# Autodesk Inventor assembly: TopAssembly
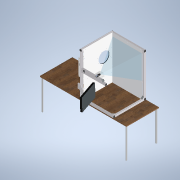
[picture p0: Inventor's stored thumbnail of the model, 180x180]
Saved by Autodesk Inventor 2020 (Build 240168000, 168)
## iProperties
Created: 2019-11-06
Part Number: TopAssembly
Document SubType Name: Assembly
Designer: nicoc
Author: nicoc
## Documents named in this file (9)
- D:\Repos\P5-AIonFPGA\cad\TopAssembly.iam
- D:\Repos\P5-AIonFPGA\cad\BasicFramework\BasicFramework.iam
- D:\Repos\P5-AIonFPGA\cad\RearPanel\RearPanel.iam
- D:\Repos\P5-AIonFPGA\cad\SidePanel\SidePanel.iam
- D:\Repos\P5-AIonFPGA\cad\Cameramounting\Cameramounting.iam
- D:\Repos\P5-AIonFPGA\cad\Table\Table.iam
- D:\Repos\P5-AIonFPGA\cad\Display\Display.iam
- D:\Repos\P5-AIonFPGA\cad\Case\Case.iam
- D:\Repos\P5-AIonFPGA\cad\Lighting\LHF300\LHF300-R2.iam
## Components (8 placed, 8 different names)
1. BasicFramework:1 [sub-assembly] — Mate:1, Flush:1, Mate:2, Mate:5, Flush:3, Mate:6, Mate:7, Flush:4, Flush:5, Mate:8, Mate:10, Flush:7, Mate:17, Flush:9, Mate:18, Flush:11
2. RearPanel:1 [sub-assembly] — Mate:1, Flush:1, Mate:2, Mate:11, Mate:14
3. SidePanel:1 [sub-assembly] — Mate:10, Flush:7, Mate:11
4. Cameramounting:1 [sub-assembly] — Mate:5, Flush:3, Mate:6, Flush:10
5. Table:1 [sub-assembly] — Mate:7, Flush:4, Flush:5
6. Display:1 [sub-assembly] — Mate:8, Mate:17, Flush:9
7. Case:1 [sub-assembly] — Mate:14
8. LHF300-R2:1 [sub-assembly] — Flush:10, Mate:18, Flush:11
## Relationships (19: Mate 11, Flush 8)
- Mate:1: BasicFramework:1 ↔ RearPanel:1
- Flush:1: BasicFramework:1 ↔ RearPanel:1
- Mate:2 (0.5 mm): BasicFramework:1 ↔ RearPanel:1
- Mate:5: BasicFramework:1 ↔ Cameramounting:1
- Flush:3: BasicFramework:1 ↔ Cameramounting:1
- Mate:6 (-664.5 mm): BasicFramework:1 ↔ Cameramounting:1
- Mate:7: BasicFramework:1 ↔ Table:1
- Flush:4: BasicFramework:1 ↔ Table:1
- Flush:5 (-300 mm): BasicFramework:1 ↔ Table:1
- Mate:8: BasicFramework:1 ↔ Display:1
- Mate:10: BasicFramework:1 ↔ SidePanel:1
- Flush:7: BasicFramework:1 ↔ SidePanel:1
- Mate:11: RearPanel:1 ↔ SidePanel:1
- Mate:14 (5 mm): RearPanel:1 ↔ Case:1
- Mate:17: BasicFramework:1 ↔ Display:1
- Flush:9: BasicFramework:1 ↔ Display:1
- Flush:10: Cameramounting:1 ↔ LHF300-R2:1
- Mate:18: BasicFramework:1 ↔ LHF300-R2:1
- Flush:11 (5 mm): BasicFramework:1 ↔ LHF300-R2:1
